# Autodesk Inventor assembly: Assembly2
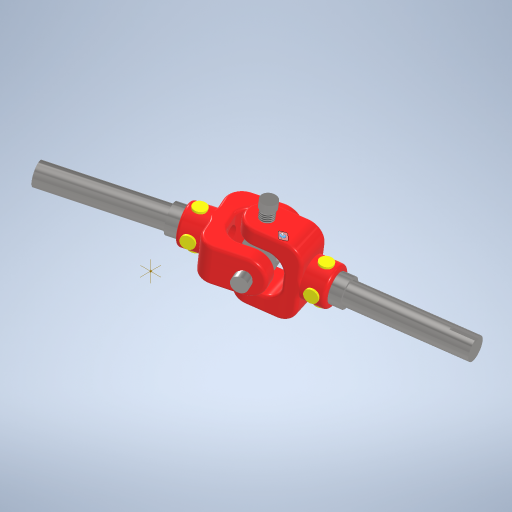
[picture p0: Inventor's stored thumbnail of the model, 512x512]
Saved by Autodesk Inventor 2024 (Build 280153000, 153)
## iProperties
Created: 2023-10-30
Part Number: Assembly2
Document SubType Name: Assembly
Designer: Admin
Author: Admin
## Documents named in this file (6)
- C:\Users\Admin\Documents\Inventor\class6.assembly\Assembly2.iam
- C:\Users\Admin\Documents\Inventor\class6.assembly\base.ipt
- C:\Users\Admin\Documents\Inventor\class6.assembly\bolt.ipt
- C:\Users\Admin\Documents\Inventor\class6.assembly\nut.ipt
- C:\Users\Admin\Documents\Inventor\class6.assembly\shaft.ipt
- C:\Users\Admin\Documents\Inventor\class6.assembly\pin.ipt
## Components (17 placed, 5 different names)
1. base:1 — Cylindrical:1, Cylindrical:2, Mate:1, Rotational:6, Rigid:1
2. bolt:1 — Cylindrical:2, Rotational:2
3. bolt:2 — Cylindrical:1, Rotational:3, Mate:1
4. nut:1 — Rotational:2, Rotational:3, Rotational:4, Rotational:5
5. base:2 — Cylindrical:4, Cylindrical:5, Rotational:7, Rigid:2
6. bolt:3 — Cylindrical:4, Rotational:4
7. bolt:4 — Cylindrical:5, Rotational:5
8. shaft:1 — Rotational:7
9. shaft:2 — Rotational:6
10. pin:1 — Rigid:1
11. pin:6
12. pin:7
13. pin:8
14. pin:5 — Rigid:2
15. pin:9
16. pin:10
17. pin:11
## Component patterns: (4 elements, first: pin:1), (4 elements, first: pin:5)
## Relationships (13: RevoluteJoint 6, CylindricalJoint 4, WeldJoint 2, Mate 1)
- Cylindrical:1: base:1 ↔ bolt:2
- Cylindrical:2: base:1 ↔ bolt:1
- Rotational:2 [RevoluteJoint] (3 mm): bolt:1 ↔ nut:1
- Rotational:3 [RevoluteJoint] (3 mm): bolt:2 ↔ nut:1
- Cylindrical:4: base:2 ↔ bolt:3
- Rotational:4 [RevoluteJoint]: nut:1 ↔ bolt:3
- Cylindrical:5: base:2 ↔ bolt:4
- Rotational:5 [RevoluteJoint]: nut:1 ↔ bolt:4
- Mate:1: base:1 ↔ bolt:2
- Rotational:6 [RevoluteJoint]: base:1 ↔ shaft:2
- Rotational:7 [RevoluteJoint]: base:2 ↔ shaft:1
- Rigid:1 [WeldJoint]: base:1 ↔ pin:1
- Rigid:2 [WeldJoint]: base:2 ↔ pin:5
